# Autodesk Inventor assembly: MTLV-S99
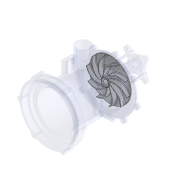
[picture p0: Inventor's stored thumbnail of the model, 180x180]
Saved by Autodesk Inventor 2020 (Build 240168000, 168)
## iProperties
Created: 2020-03-28
Part Number: MTLV-S99
Document SubType Name: Assembly
Designer: John K
Description: TURBINE ASSEMBLY
Author: John K
## Documents named in this file (4)
- C:\GrabCAD\MTL Ventilator Design\MTLV\Subassemblies\MTLV-S99.iam
- C:\GrabCAD\MTL Ventilator Design\MTLV\Manufactured Parts\MTLV-P01.ipt
- C:\GrabCAD\MTL Ventilator Design\MTLV\Manufactured Parts\MTLV-P02.ipt
- C:\GrabCAD\MTL Ventilator Design\MTLV\Manufactured Parts\MTLV-P18.ipt
## Components (3 placed, 3 different names)
1. MTLV-P01:1 — Mate:14, Mate:15
2. MTLV-P02:1 — Mate:14, Mate:15, Mate:16, Mate:17
3. MTLV-P18:1 — Mate:16, Mate:17
## Relationships (4: Mate 4)
- Mate:14: MTLV-P01:1 ↔ MTLV-P02:1
- Mate:15: MTLV-P01:1 ↔ MTLV-P02:1
- Mate:16 (0.3 mm): MTLV-P02:1 ↔ MTLV-P18:1
- Mate:17: MTLV-P02:1 ↔ MTLV-P18:1
